# Autodesk Inventor assembly: yaw_unit_mir1
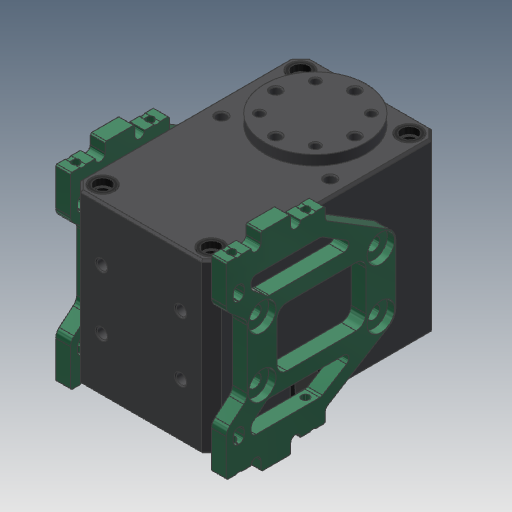
[picture p0: Inventor's stored thumbnail of the model, 512x512]
Saved by Autodesk Inventor 2019.4 (Build 234330000, 330)
## iProperties
Created: 2018-08-06
Part Number: yaw_unit_mir1
Material: 一般
Document SubType Name: Assembly
Designer: y6tada
Mass: 47.0989 g
Surface Area: 177.769 cm^2
Volume: 47.0989 cm^3
Density: 1 g/cm^3
Author: student
## Documents named in this file (4)
- C:\Workspace\HaptHexa\Hardware\Inventor\Thorax\yaw_unit\yaw_unit_mir1.iam
- C:\Workspace\HaptHexa\Hardware\Inventor\Thorax\yaw_unit\yaw_servo_side_mir3.ipt
- C:\Workspace\HaptHexa\Hardware\Inventor\Thorax\yaw_unit\yaw_servo_side_mir1_mir1.ipt
- C:\Workspace\HaptHexa\Hardware\Inventor\X430\XL-430.iam
## Components (3 placed, 3 different names)
1. XL-430:1 [sub-assembly] — メイト:2, メイト:3, メイト:4, メイト:5, メイト:6, メイト:7
2. yaw_servo_side_mir3:1 — メイト:5, メイト:6, メイト:7
3. yaw_servo_side_mir1_mir1:1 — メイト:2, メイト:3, メイト:4
## Relationships (9: Mate 7, Flush 2)
- [Mate]: XL-430:1
- [Flush]: XL-430:1
- [Flush]: XL-430:1
- メイト:2 [Mate]: XL-430:1 ↔ yaw_servo_side_mir1_mir1:1
- メイト:3 [Mate]: XL-430:1 ↔ yaw_servo_side_mir1_mir1:1
- メイト:4 [Mate]: XL-430:1 ↔ yaw_servo_side_mir1_mir1:1
- メイト:5 [Mate]: XL-430:1 ↔ yaw_servo_side_mir3:1
- メイト:6 [Mate]: XL-430:1 ↔ yaw_servo_side_mir3:1
- メイト:7 [Mate]: XL-430:1 ↔ yaw_servo_side_mir3:1
